# Autodesk Inventor assembly: 2inShooters
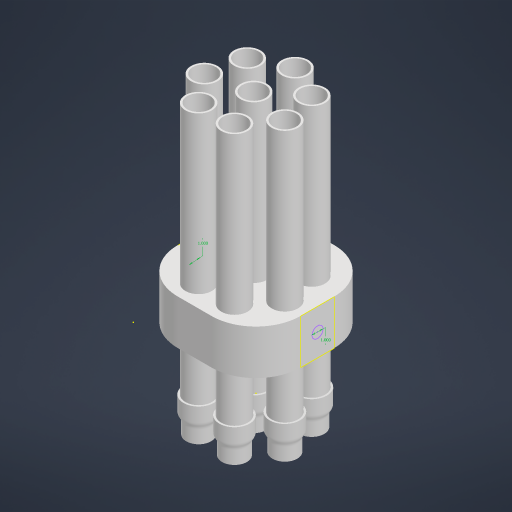
[picture p0: Inventor's stored thumbnail of the model, 512x512]
Saved by Autodesk Inventor 2023 (Build 270158000, 158)
## iProperties
Created: 2022-06-22
Part Number: 2inShooters
Document SubType Name: Assembly
Designer: timmy
Author: timmy
## Documents named in this file (3)
- R:\Inventor\RoboCatz\T-Shirt\Rev2-Better\2inShooters.iam
- R:\Inventor\RoboCatz\T-Shirt\Rev2-Better\ShooterMount-1in.ipt
- R:\Inventor\RoboCatz\T-Shirt\Rev2-Better\2inShooterpipe.iam
## Components (9 placed, 2 different names)
1. ShooterMount-1in:1 — Mate:1, Mate:2, Mate:3, Mate:4, Mate:5, Mate:6, Mate:7, Mate:8
2. 2inShooterpipe:1 [sub-assembly] — Mate:4, Flush:4
3. 2inShooterpipe:2 [sub-assembly] — Mate:3, Flush:3
4. 2inShooterpipe:3 [sub-assembly] — Mate:1, Flush:2
5. 2inShooterpipe:4 [sub-assembly] — Mate:6, Flush:6
6. 2inShooterpipe:5 [sub-assembly] — Mate:7, Flush:7
7. 2inShooterpipe:6 [sub-assembly] — Mate:8, Flush:1, Flush:8
8. 2inShooterpipe:7 [sub-assembly] — Mate:5, Flush:5
9. 2inShooterpipe:8 [sub-assembly] — Mate:2, Flush:1, Flush:2, Flush:3, Flush:4, Flush:5, Flush:6, Flush:7, Flush:8
## Relationships (16: Mate 8, Flush 8)
- Mate:1: ShooterMount-1in:1 ↔ 2inShooterpipe:3
- Mate:2: ShooterMount-1in:1 ↔ 2inShooterpipe:8
- Mate:3: ShooterMount-1in:1 ↔ 2inShooterpipe:2
- Mate:4: ShooterMount-1in:1 ↔ 2inShooterpipe:1
- Mate:5: ShooterMount-1in:1 ↔ 2inShooterpipe:7
- Mate:6: ShooterMount-1in:1 ↔ 2inShooterpipe:4
- Mate:7: ShooterMount-1in:1 ↔ 2inShooterpipe:5
- Mate:8: ShooterMount-1in:1 ↔ 2inShooterpipe:6
- Flush:1: 2inShooterpipe:6 ↔ 2inShooterpipe:8
- Flush:2: 2inShooterpipe:3 ↔ 2inShooterpipe:8
- Flush:3: 2inShooterpipe:2 ↔ 2inShooterpipe:8
- Flush:4: 2inShooterpipe:1 ↔ 2inShooterpipe:8
- Flush:5: 2inShooterpipe:7 ↔ 2inShooterpipe:8
- Flush:6: 2inShooterpipe:4 ↔ 2inShooterpipe:8
- Flush:7: 2inShooterpipe:5 ↔ 2inShooterpipe:8
- Flush:8: 2inShooterpipe:6 ↔ 2inShooterpipe:8
